# Autodesk Inventor assembly: GE-13018
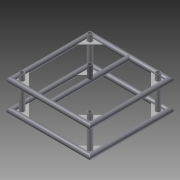
[picture p0: Inventor's stored thumbnail of the model, 180x180]
Saved by Autodesk Inventor 2013 (Build 170138000, 138)
## iProperties
Created: 2013-01-05
Part Number: GE-13018
Document SubType Name: Assembly
Designer: Phillip
Author: Phillip
## Documents named in this file (4)
- E:\Data Folder\FIRST 2013\FIRST KOP\FIRST Arena 2013\Pyramid\GE-13018.iam
- E:\Data Folder\FIRST 2013\FIRST KOP\FIRST Arena 2013\Pyramid\GE-13018-04.iam
- E:\Data Folder\FIRST 2013\FIRST KOP\FIRST Arena 2013\Pyramid\GE-13018-05.ipt
- E:\Data Folder\FIRST 2013\FIRST KOP\FIRST Arena 2013\Pyramid\GE-13018-01.ipt
## Components (14 placed, 3 different names)
1. GE-13018-04:1 [sub-assembly] — Tangent:1, Tangent:2, Tangent:3, Tangent:4, Mate:1, Mate:2, Tangent:5, Tangent:6, Mate:3, Tangent:7, Mate:4, Tangent:8, Tangent:9, Tangent:18, Mate:13, Mate:14, Mate:15, Mate:16
2. GE-13018-04:2 [sub-assembly] — Mate:5, Tangent:10, Tangent:11, Mate:6, Tangent:12, Tangent:13, Mate:7, Tangent:14, Tangent:15, Mate:8, Tangent:16, Tangent:17
3. GE-13018-05:1 — Tangent:1, Tangent:2, Mate:1
4. GE-13018-05:2 — Tangent:3, Tangent:4, Mate:2
5. GE-13018-05:3 — Tangent:5, Mate:3, Tangent:7, Flush:1
6. GE-13018-05:4 — Mate:7, Tangent:14, Tangent:15, Flush:1
7. GE-13018-05:5 — Mate:8, Tangent:16, Tangent:17, Mate:10
8. GE-13018-05:6 — Mate:4, Tangent:8, Tangent:9, Mate:10, Insert:2, Mate:11, Angle:2
9. GE-13018-05:7 — Mate:5, Tangent:10, Tangent:11
10. GE-13018-05:8 — Tangent:6, Mate:6, Tangent:12, Tangent:13
11. GE-13018-01:2 — Insert:2, Mate:12
12. GE-13018-01:3
13. GE-13018-01:4
14. GE-13018-01:5
## Component patterns: (4 elements, first: GE-13018-01:2)
## Relationships (37: Tangent 18, Mate 15, Angle 2, Insert 1, Flush 1)
- Tangent:1: GE-13018-04:1 ↔ GE-13018-05:1
- Tangent:2: GE-13018-04:1 ↔ GE-13018-05:1
- Tangent:3: GE-13018-04:1 ↔ GE-13018-05:2
- Tangent:4: GE-13018-04:1 ↔ GE-13018-05:2
- Mate:1: GE-13018-04:1 ↔ GE-13018-05:1
- Mate:2: GE-13018-04:1 ↔ GE-13018-05:2
- Tangent:5: GE-13018-04:1 ↔ GE-13018-05:3
- Tangent:6: GE-13018-04:1 ↔ GE-13018-05:8
- Mate:3: GE-13018-04:1 ↔ GE-13018-05:3
- Tangent:7: GE-13018-04:1 ↔ GE-13018-05:3
- Mate:4: GE-13018-04:1 ↔ GE-13018-05:6
- Tangent:8: GE-13018-04:1 ↔ GE-13018-05:6
- Tangent:9: GE-13018-04:1 ↔ GE-13018-05:6
- Mate:5: GE-13018-04:2 ↔ GE-13018-05:7
- Tangent:10: GE-13018-04:2 ↔ GE-13018-05:7
- Tangent:11: GE-13018-04:2 ↔ GE-13018-05:7
- Mate:6: GE-13018-04:2 ↔ GE-13018-05:8
- Tangent:12: GE-13018-04:2 ↔ GE-13018-05:8
- Tangent:13: GE-13018-04:2 ↔ GE-13018-05:8
- Mate:7: GE-13018-04:2 ↔ GE-13018-05:4
- Tangent:14: GE-13018-04:2 ↔ GE-13018-05:4
- Tangent:15: GE-13018-04:2 ↔ GE-13018-05:4
- Mate:8: GE-13018-04:2 ↔ GE-13018-05:5
- Tangent:16: GE-13018-04:2 ↔ GE-13018-05:5
- Tangent:17: GE-13018-04:2 ↔ GE-13018-05:5
- Mate:10: GE-13018-05:5 ↔ GE-13018-05:6
- Insert:2 (-50.8 mm): GE-13018-05:6 ↔ GE-13018-01:2
- Mate:11: GE-13018-05:6
- Angle:2 (0 deg): GE-13018-05:6
- Mate:12: GE-13018-01:2
- Angle:3 (0 deg)
- Tangent:18: GE-13018-04:1
- Mate:13: GE-13018-04:1
- Mate:14: GE-13018-04:1
- Mate:15: GE-13018-04:1
- Mate:16: GE-13018-04:1
- Flush:1 (-215.9 mm): GE-13018-05:3 ↔ GE-13018-05:4
